# Autodesk Inventor assembly: Final AssemblyV5
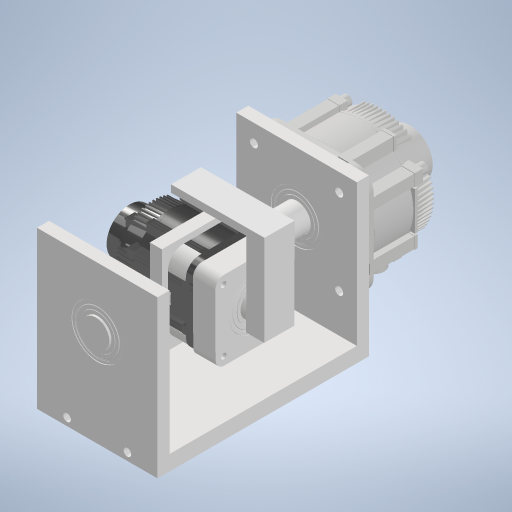
[picture p0: Inventor's stored thumbnail of the model, 512x512]
Saved by Autodesk Inventor 2024 (Build 280153000, 153)
## iProperties
Created: 2024-02-08
Part Number: Final AssemblyV5
Document SubType Name: Assembly
Designer: yusuf
Author: yusuf
## Documents named in this file (9)
- C:\Users\yusuf\Documents\DodgeBot\design\hardware\CAD_FILES\Final AssemblyV5.iam
- C:\Users\yusuf\Documents\DodgeBot\design\hardware\CAD_FILES\YASKAWA_USA_SGM7G30A6A61\AIS2024\SGM7G-30A6A61.iam
- C:\Users\yusuf\Documents\DodgeBot\design\hardware\CAD_FILES\FrontPlateV2.ipt
- C:\Users\yusuf\Documents\DodgeBot\design\hardware\CAD_FILES\SGM7G_20AxA61\SGM7G-20xxA61\ProE\SGM7G-20__a61_ProE\ProE\sgm7g_20__a61\sgm7g_20__a61.iam
- C:\Users\yusuf\Documents\DodgeBot\design\hardware\CAD_FILES\145100992-9-skf_bearing_6209-2z_2\skf_bearing_6209-2z_2.iam
- C:\Users\yusuf\Documents\DodgeBot\design\hardware\CAD_FILES\FloorMount.ipt
- C:\Users\yusuf\Documents\DodgeBot\design\hardware\CAD_FILES\FloorMountFacePlate.ipt
- C:\Users\yusuf\Documents\DodgeBot\design\hardware\CAD_FILES\EndEffectorMotorAdapter.ipt
- C:\Users\yusuf\Documents\DodgeBot\design\hardware\CAD_FILES\EndEffectorMotorAdapterOLD.ipt
## Components (10 placed, 8 different names)
1. SGM7G-30A6A61:1 [sub-assembly] — Rigid:4, Rotational:4
2. FrontPlateV2:1 — Rigid:1, Rotational:4
3. sgm7g_20__a61:1 [sub-assembly] — Rigid:1, Rotational:6, Rigid:5
4. skf_bearing_6209-2z_2:1 [sub-assembly] — Rotational:7
5. skf_bearing_6209-2z_2:2 [sub-assembly] — Rotational:2
6. FloorMount:1 — Rotational:2, Rigid:4, Rigid:6
7. FloorMountFacePlate:1 — Rotational:7, Rigid:6
8. EndEffectorMotorAdapter:1 — Rotational:5, Rigid:5
9. skf_bearing_6209-2z_2:3 [sub-assembly] — Rotational:5
10. EndEffectorMotorAdapterOLD:1 — Rotational:6
## Relationships (9: RevoluteJoint 5, WeldJoint 4)
- Rigid:1 [WeldJoint] (-109 mm): FrontPlateV2:1 ↔ sgm7g_20__a61:1
- Rotational:2 [RevoluteJoint]: skf_bearing_6209-2z_2:2 ↔ FloorMount:1
- Rigid:4 [WeldJoint]: SGM7G-30A6A61:1 ↔ FloorMount:1
- Rotational:4 [RevoluteJoint]: SGM7G-30A6A61:1 ↔ FrontPlateV2:1
- Rotational:5 [RevoluteJoint]: EndEffectorMotorAdapter:1 ↔ skf_bearing_6209-2z_2:3
- Rotational:6 [RevoluteJoint] (-20 mm): sgm7g_20__a61:1 ↔ EndEffectorMotorAdapterOLD:1
- Rotational:7 [RevoluteJoint]: skf_bearing_6209-2z_2:1 ↔ FloorMountFacePlate:1
- Rigid:5 [WeldJoint]: sgm7g_20__a61:1 ↔ EndEffectorMotorAdapter:1
- Rigid:6 [WeldJoint]: FloorMount:1 ↔ FloorMountFacePlate:1
